# Autodesk Inventor assembly: Test tube rack
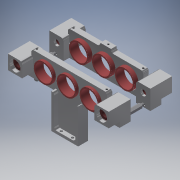
[picture p0: Inventor's stored thumbnail of the model, 180x180]
Saved by Autodesk Inventor 2017 (Build 210142000, 142)
## iProperties
Created: 2016-12-06
Part Number: Test tube rack
Document SubType Name: Assembly
Designer: qupec
Author: qupec
## Documents named in this file (10)
- C:\UMD\BPP\ROCKSAT X\STAR\CAD\Mechanical\Full payload assembly\Subsystems\Test Tube Rack\Test tube rack.iam
- C:\UMD\BPP\ROCKSAT X\STAR\CAD\Mechanical\Full payload assembly\Subsystems\Test Tube Rack\Test Tube Holder with Camera.ipt
- C:\UMD\BPP\ROCKSAT X\STAR\CAD\Mechanical\Full payload assembly\Subsystems\Test Tube Rack\Tube Rubber.ipt
- C:\UMD\BPP\ROCKSAT X\STAR\CAD\Mechanical\Full payload assembly\Subsystems\Test Tube Rack\Test Tube Holder.ipt
- C:\UMD\BPP\ROCKSAT X\STAR\CAD\Mechanical\Full payload assembly\Subsystems\Test Tube Rack\Bottom Test Tube Holder.ipt
- C:\UMD\BPP\ROCKSAT X\STAR\CAD\Mechanical\Full payload assembly\Subsystems\Test Tube Rack\Top Test Tube Holder.ipt
- C:\UMD\BPP\ROCKSAT X\STAR\CAD\Mechanical\Full payload assembly\Subsystems\Test Tube Rack\Self-Aligning PTFE Bearing.ipt
- C:\UMD\BPP\ROCKSAT X\STAR\CAD\Mechanical\Full payload assembly\Subsystems\Fasteners\Num4 Narrow Split Washer.ipt
- C:\UMD\BPP\ROCKSAT X\STAR\CAD\Mechanical\Full payload assembly\Subsystems\Fasteners\4-40 1in Socket Screw.ipt
- C:\UMD\BPP\ROCKSAT X\STAR\CAD\Mechanical\Full payload assembly\Subsystems\Fasteners\.75 in Standoff.ipt
## Components (20 placed, 9 different names)
1. Test Tube Holder:1 — Mate:61, Mate:75, Mate:76, Mate:77, Mate:78
2. Bottom Test Tube Holder:1 — Mate:7, Mate:8, Mate:9, Mate:61
3. Tube Rubber:1
4. Tube Rubber:2
5. Tube Rubber:3 — Mate:8, Mate:82, Flush:16, Flush:17
6. Tube Rubber:4 — Mate:9
7. Tube Rubber:5 — Mate:7, Mate:83, Flush:15, Flush:16
8. Tube Rubber:6 — Mate:81, Flush:17
9. Test Tube Holder with Camera:1 — Mate:60, Mate:70, Flush:14, Mate:71, Mate:72, Mate:73, Mate:74, Mate:79, Mate:80, Mate:81, Flush:15, Mate:84, Mate:85, Mate:86, Mate:87, Mate:88, Mate:89, Mate:90, Mate:91, Mate:92, Mate:93, Mate:94, Mate:95
10. Top Test Tube Holder:1 — Mate:60, Mate:79, Mate:80, Mate:82, Mate:83
11. Self-Aligning PTFE Bearing:1 — Mate:71, Mate:74
12. Self-Aligning PTFE Bearing:2 — Mate:76, Mate:77
13. Self-Aligning PTFE Bearing:3 — Mate:75, Mate:78
14. Self-Aligning PTFE Bearing:4 — Mate:72, Mate:73
15. Num4 Narrow Split Washer:1 — Mate:84, Mate:85
16. Num4 Narrow Split Washer:2 — Mate:86, Mate:87
17. 4-40 1in Socket Screw:1 — Mate:88, Mate:90
18. 4-40 1in Socket Screw:2 — Mate:89, Mate:91
19. .75 in Standoff:1 — Mate:92, Mate:93
20. .75 in Standoff:2 — Mate:94, Mate:95
## Relationships (35: Mate 31, Flush 4)
- Mate:7: Bottom Test Tube Holder:1 ↔ Tube Rubber:5
- Mate:8: Bottom Test Tube Holder:1 ↔ Tube Rubber:3
- Mate:9: Bottom Test Tube Holder:1 ↔ Tube Rubber:4
- Mate:60: Test Tube Holder with Camera:1 ↔ Top Test Tube Holder:1
- Mate:61: Test Tube Holder:1 ↔ Bottom Test Tube Holder:1
- Mate:70: Test Tube Holder with Camera:1
- Flush:14: Test Tube Holder with Camera:1
- Mate:71: Test Tube Holder with Camera:1 ↔ Self-Aligning PTFE Bearing:1
- Mate:72: Test Tube Holder with Camera:1 ↔ Self-Aligning PTFE Bearing:4
- Mate:73: Test Tube Holder with Camera:1 ↔ Self-Aligning PTFE Bearing:4
- Mate:74: Test Tube Holder with Camera:1 ↔ Self-Aligning PTFE Bearing:1
- Mate:75: Test Tube Holder:1 ↔ Self-Aligning PTFE Bearing:3
- Mate:76: Test Tube Holder:1 ↔ Self-Aligning PTFE Bearing:2
- Mate:77: Test Tube Holder:1 ↔ Self-Aligning PTFE Bearing:2
- Mate:78: Test Tube Holder:1 ↔ Self-Aligning PTFE Bearing:3
- Mate:79: Test Tube Holder with Camera:1 ↔ Top Test Tube Holder:1
- Mate:80: Test Tube Holder with Camera:1 ↔ Top Test Tube Holder:1
- Mate:81: Tube Rubber:6 ↔ Test Tube Holder with Camera:1
- Mate:82: Tube Rubber:3 ↔ Top Test Tube Holder:1
- Mate:83: Tube Rubber:5 ↔ Top Test Tube Holder:1
- Flush:15: Tube Rubber:5 ↔ Test Tube Holder with Camera:1
- Flush:16: Tube Rubber:3 ↔ Tube Rubber:5
- Flush:17: Tube Rubber:3 ↔ Tube Rubber:6
- Mate:84: Test Tube Holder with Camera:1 ↔ Num4 Narrow Split Washer:1
- Mate:85: Test Tube Holder with Camera:1 ↔ Num4 Narrow Split Washer:1
- Mate:86: Test Tube Holder with Camera:1 ↔ Num4 Narrow Split Washer:2
- Mate:87: Test Tube Holder with Camera:1 ↔ Num4 Narrow Split Washer:2
- Mate:88: Test Tube Holder with Camera:1 ↔ 4-40 1in Socket Screw:1
- Mate:89: Test Tube Holder with Camera:1 ↔ 4-40 1in Socket Screw:2
- Mate:90: Test Tube Holder with Camera:1 ↔ 4-40 1in Socket Screw:1
- Mate:91: Test Tube Holder with Camera:1 ↔ 4-40 1in Socket Screw:2
- Mate:92: Test Tube Holder with Camera:1 ↔ .75 in Standoff:1
- Mate:93: Test Tube Holder with Camera:1 ↔ .75 in Standoff:1
- Mate:94: Test Tube Holder with Camera:1 ↔ .75 in Standoff:2
- Mate:95: Test Tube Holder with Camera:1 ↔ .75 in Standoff:2
